# Autodesk Inventor assembly: Donna
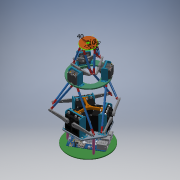
[picture p0: Inventor's stored thumbnail of the model, 180x180]
Saved by Autodesk Inventor 2018.2 (Build 222227000, 227)
## iProperties
Created: 2018-02-19
Part Number: Donna
Material: Generisch
Document SubType Name: Assembly
Designer: JochenAlt
Author: JochenAlt
## Documents named in this file (9)
- D:\Projects\Donna\CAD\Donna.iam
- D:\Projects\Donna\CAD\Base-Plate.ipt
- D:\Projects\Donna\CAD\Stewart-Platform.iam
- D:\Projects\Donna\CAD\Base-Stewart-Connector.ipt
- D:\Projects\Donna\CAD\ODroid C2\ODroid C2.iam
- D:\Projects\Donna\CAD\Teensy 3.5-3.6\Teensy.iam
- D:\Projects\Donna\CAD\Servo-Arm-20mm-Ball-Joint.iam
- D:\Projects\Donna\CAD\Ball-Joint-Rod-Small.iam
- D:\Projects\Donna\CAD\Stewart-Head.iam
## Components (20 placed, 8 different names)
1. Base-Plate:1 — Passend:1, Passend:2, Passend:3, Passend:4, Passend:5, Passend:6, Winkel:1, Passend:10, Winkel:3
2. Stewart Platform Inside:1 [sub-assembly] — Passend:7, Passend:8, Passend:9, Winkel:2, Passend:11, Passend:12, Passend:13, Passend:14, Passend:15, Passend:16, Passend:17, Passend:18, Passend:19, Passend:20, Passend:21, Passend:22
3. Base-Stewart-Connector:1 — Passend:2, Passend:6, Passend:9
4. Base-Stewart-Connector:2 — Passend:3, Passend:4, Passend:8
5. Base-Stewart-Connector:3 — Passend:1, Passend:5, Passend:7
6. ODroid C2:1 [sub-assembly] — Winkel:1, Winkel:2, Passend:10, Winkel:4
7. Teensy:1 [sub-assembly] — Winkel:3, Winkel:4
8. Servo-Arm-20mm-Ball-Joint:1 [sub-assembly] — Passend:11, Passend:22, Passend:28
9. Servo-Arm-20mm-Ball-Joint:2 [sub-assembly] — Passend:12, Passend:21, Passend:26
10. Servo-Arm-20mm-Ball-Joint:3 [sub-assembly] — Passend:13, Passend:18, Passend:23
11. Servo-Arm-20mm-Ball-Joint:4 [sub-assembly] — Passend:16, Passend:20, Passend:27
12. Servo-Arm-20mm-Ball-Joint:5 [sub-assembly] — Passend:14, Passend:17, Passend:24
13. Servo-Arm-20mm-Ball-Joint:6 [sub-assembly] — Passend:15, Passend:19, Passend:25
14. Ball Joint Rod Small:1 [sub-assembly] — Passend:23, Passend:32
15. Ball Joint Rod Small:2 [sub-assembly] — Passend:24, Passend:31
16. Ball Joint Rod Small:3 [sub-assembly] — Passend:25, Passend:30
17. Ball Joint Rod Small:4 [sub-assembly] — Passend:27, Passend:29
18. Ball Joint Rod Small:5 [sub-assembly] — Passend:28, Passend:33
19. Ball Joint Rod Small:6 [sub-assembly] — Passend:26, Passend:34
20. Stewart-Head:1 [sub-assembly] — Passend:29, Passend:30, Passend:31, Passend:32, Passend:33, Passend:34
## Relationships (38: Mate 34, Angle 4)
- Passend:1 [Mate]: Base-Plate:1 ↔ Base-Stewart-Connector:3
- Passend:2 [Mate]: Base-Plate:1 ↔ Base-Stewart-Connector:1
- Passend:3 [Mate]: Base-Plate:1 ↔ Base-Stewart-Connector:2
- Passend:4 [Mate]: Base-Plate:1 ↔ Base-Stewart-Connector:2
- Passend:5 [Mate]: Base-Plate:1 ↔ Base-Stewart-Connector:3
- Passend:6 [Mate]: Base-Plate:1 ↔ Base-Stewart-Connector:1
- Passend:7 [Mate]: Stewart Platform Inside:1 ↔ Base-Stewart-Connector:3
- Passend:8 [Mate]: Stewart Platform Inside:1 ↔ Base-Stewart-Connector:2
- Passend:9 [Mate]: Stewart Platform Inside:1 ↔ Base-Stewart-Connector:1
- Winkel:1 [Angle] (180 deg): Base-Plate:1 ↔ ODroid C2:1
- Winkel:2 [Angle] (0 deg): Stewart Platform Inside:1 ↔ ODroid C2:1
- Passend:10 [Mate] (5 mm): Base-Plate:1 ↔ ODroid C2:1
- Winkel:3 [Angle] (0 deg): Base-Plate:1 ↔ Teensy:1
- Winkel:4 [Angle] (180 deg): ODroid C2:1 ↔ Teensy:1
- Passend:11 [Mate]: Stewart Platform Inside:1 ↔ Servo-Arm-20mm-Ball-Joint:1
- Passend:12 [Mate]: Stewart Platform Inside:1 ↔ Servo-Arm-20mm-Ball-Joint:2
- Passend:13 [Mate]: Stewart Platform Inside:1 ↔ Servo-Arm-20mm-Ball-Joint:3
- Passend:14 [Mate]: Stewart Platform Inside:1 ↔ Servo-Arm-20mm-Ball-Joint:5
- Passend:15 [Mate]: Stewart Platform Inside:1 ↔ Servo-Arm-20mm-Ball-Joint:6
- Passend:16 [Mate]: Stewart Platform Inside:1 ↔ Servo-Arm-20mm-Ball-Joint:4
- Passend:17 [Mate]: Stewart Platform Inside:1 ↔ Servo-Arm-20mm-Ball-Joint:5
- Passend:18 [Mate]: Stewart Platform Inside:1 ↔ Servo-Arm-20mm-Ball-Joint:3
- Passend:19 [Mate]: Stewart Platform Inside:1 ↔ Servo-Arm-20mm-Ball-Joint:6
- Passend:20 [Mate]: Stewart Platform Inside:1 ↔ Servo-Arm-20mm-Ball-Joint:4
- Passend:21 [Mate]: Stewart Platform Inside:1 ↔ Servo-Arm-20mm-Ball-Joint:2
- Passend:22 [Mate]: Stewart Platform Inside:1 ↔ Servo-Arm-20mm-Ball-Joint:1
- Passend:23 [Mate]: Servo-Arm-20mm-Ball-Joint:3 ↔ Ball Joint Rod Small:1
- Passend:24 [Mate]: Servo-Arm-20mm-Ball-Joint:5 ↔ Ball Joint Rod Small:2
- Passend:25 [Mate]: Servo-Arm-20mm-Ball-Joint:6 ↔ Ball Joint Rod Small:3
- Passend:26 [Mate]: Servo-Arm-20mm-Ball-Joint:2 ↔ Ball Joint Rod Small:6
- Passend:27 [Mate]: Servo-Arm-20mm-Ball-Joint:4 ↔ Ball Joint Rod Small:4
- Passend:28 [Mate]: Servo-Arm-20mm-Ball-Joint:1 ↔ Ball Joint Rod Small:5
- Passend:29 [Mate]: Ball Joint Rod Small:4 ↔ Stewart-Head:1
- Passend:30 [Mate]: Ball Joint Rod Small:3 ↔ Stewart-Head:1
- Passend:31 [Mate]: Ball Joint Rod Small:2 ↔ Stewart-Head:1
- Passend:32 [Mate]: Ball Joint Rod Small:1 ↔ Stewart-Head:1
- Passend:33 [Mate]: Ball Joint Rod Small:5 ↔ Stewart-Head:1
- Passend:34 [Mate]: Ball Joint Rod Small:6 ↔ Stewart-Head:1
